# Autodesk Inventor assembly: Tamale - V1p5p2
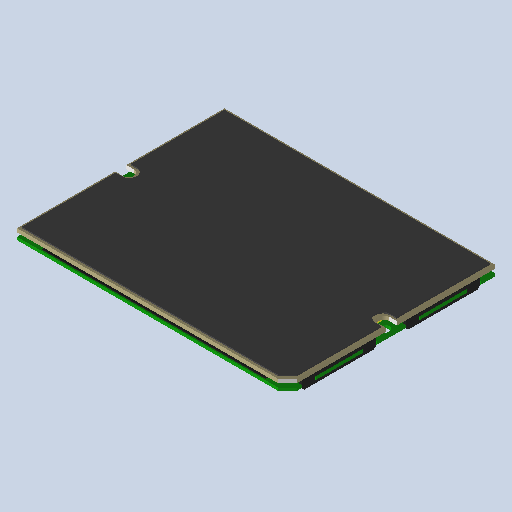
[picture p0: Inventor's stored thumbnail of the model, 512x512]
Saved by Autodesk Inventor 2025 (Build 290162000, 162)
## iProperties
Created: 2023-01-11
Part Number: Tamale - V1p5p2
Document SubType Name: Assembly
Designer: Caleb
Author: Caleb
## Documents named in this file (8)
- C:\Users\cfang\Desktop\nebraska-silicon-lab\Hardware\ETL\modules\tamale v1.5\Tamale - V1p5p2.iam
- C:\Users\cfang\Desktop\nebraska-silicon-lab\Hardware\ETL\modules\tamale v1.5\Sensor Placement Film.ipt
- C:\Users\cfang\Desktop\nebraska-silicon-lab\Hardware\ETL\modules\tamale v1.5\BBM.iam
- C:\Users\cfang\Desktop\nebraska-silicon-lab\Hardware\ETL\modules\tamale v1.5\Coverplate Film.ipt
- C:\Users\cfang\Desktop\nebraska-silicon-lab\Hardware\ETL\modules\tamale v1.5\Baseplate v1.5.1.ipt
- C:\Users\cfang\Desktop\nebraska-silicon-lab\Hardware\ETL\modules\tamale v1.5\Thermal Pad.ipt
- C:\Users\cfang\Desktop\nebraska-silicon-lab\Hardware\ETL\modules\tamale v1.5\Module PCB V1b\Module PCB V1b.ipt
- C:\Users\cfang\Desktop\nebraska-silicon-lab\Hardware\ETL\modules\tamale v1.5\insert spacer - v2.ipt
## Components (13 placed, 7 different names)
1. Sensor Placement Film:1 — Mate:2, Mate:3, Mate:4, Mate:5, Flush:3, Flush:8, Mate:23
2. BBM:1 [sub-assembly] — Mate:2, Flush:4, Mate:6, Flush:6
3. BBM:2 [sub-assembly] — Mate:5, Flush:3, Flush:4, Mate:6, Mate:7, Flush:5, Flush:8, Mate:8
4. BBM:3 [sub-assembly] — Mate:4, Flush:6, Flush:7
5. BBM:4 [sub-assembly] — Mate:3, Mate:7, Flush:5, Flush:7, Flush:9
6. Coverplate Film:1 — Mate:8, Flush:9, Mate:9
7. Baseplate v1.5.1:1 — Mate:9, Mate:22, Flush:12, Flush:13, Flush:14, Flush:15
8. Thermal Pad:1 — Mate:22, Flush:12, Flush:13
9. Module PCB V1b:1 — Mate:23, Flush:14, Flush:15, Mate:24, Mate:25, Mate:26, Mate:27, Mate:28, Mate:29, Mate:30, Mate:31, Mate:32, Mate:33, Mate:34, Mate:35
10. insert spacer - v2:1 — Mate:24, Mate:25, Mate:26
11. insert spacer - v2:2 — Mate:27, Mate:28, Mate:29
12. insert spacer - v2:3 — Mate:30, Mate:31, Mate:32
13. insert spacer - v2:4 — Mate:33, Mate:34, Mate:35
## Relationships (33: Mate 22, Flush 11)
- Mate:2: Sensor Placement Film:1 ↔ BBM:1
- Mate:3: Sensor Placement Film:1 ↔ BBM:4
- Mate:4: Sensor Placement Film:1 ↔ BBM:3
- Mate:5: Sensor Placement Film:1 ↔ BBM:2
- Flush:3 (0.5 mm): Sensor Placement Film:1 ↔ BBM:2
- Flush:4: BBM:1 ↔ BBM:2
- Mate:6 (0.2 mm): BBM:1 ↔ BBM:2
- Mate:7 (0.2 mm): BBM:2 ↔ BBM:4
- Flush:5: BBM:2 ↔ BBM:4
- Flush:6: BBM:1 ↔ BBM:3
- Flush:7: BBM:3 ↔ BBM:4
- Flush:8 (0.5 mm): Sensor Placement Film:1 ↔ BBM:2
- Mate:8: BBM:2 ↔ Coverplate Film:1
- Flush:9 (0.5 mm): BBM:4 ↔ Coverplate Film:1
- Mate:9: Coverplate Film:1 ↔ Baseplate v1.5.1:1
- Mate:22: Baseplate v1.5.1:1 ↔ Thermal Pad:1
- Flush:12 (0.5 mm): Baseplate v1.5.1:1 ↔ Thermal Pad:1
- Flush:13 (0.5 mm): Baseplate v1.5.1:1 ↔ Thermal Pad:1
- Mate:23: Sensor Placement Film:1 ↔ Module PCB V1b:1
- Flush:14: Baseplate v1.5.1:1 ↔ Module PCB V1b:1
- Flush:15: Baseplate v1.5.1:1 ↔ Module PCB V1b:1
- Mate:24: Module PCB V1b:1 ↔ insert spacer - v2:1
- Mate:25: Module PCB V1b:1 ↔ insert spacer - v2:1
- Mate:26: Module PCB V1b:1 ↔ insert spacer - v2:1
- Mate:27: Module PCB V1b:1 ↔ insert spacer - v2:2
- Mate:28: Module PCB V1b:1 ↔ insert spacer - v2:2
- Mate:29: Module PCB V1b:1 ↔ insert spacer - v2:2
- Mate:30: Module PCB V1b:1 ↔ insert spacer - v2:3
- Mate:31: Module PCB V1b:1 ↔ insert spacer - v2:3
- Mate:32: Module PCB V1b:1 ↔ insert spacer - v2:3
- Mate:33: Module PCB V1b:1 ↔ insert spacer - v2:4
- Mate:34: Module PCB V1b:1 ↔ insert spacer - v2:4
- Mate:35: Module PCB V1b:1 ↔ insert spacer - v2:4
